# Autodesk Inventor assembly: 脚クランク1
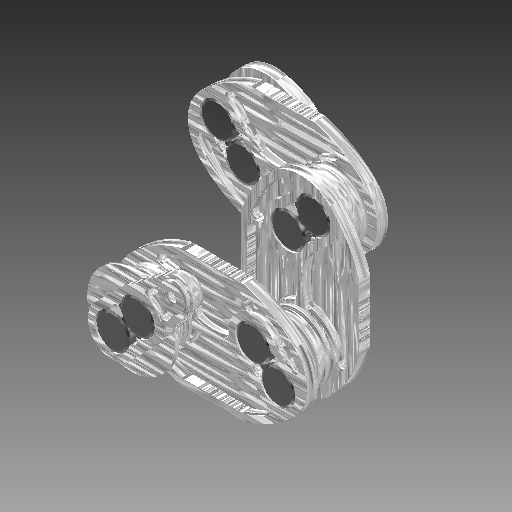
[picture p0: Inventor's stored thumbnail of the model, 512x512]
Saved by Autodesk Inventor 2020 (Build 240168000, 168)
## iProperties
Created: 2019-07-23
Part Number: 脚クランク1
Document SubType Name: Assembly
Designer: 雪村
Mass: 36.597 g
Surface Area: 166.088 cm^2
Volume: 9.97598 cm^3
Density: 3.66852 g/cm^3
Author: 雪村
## Documents named in this file (7)
- C:\Users\white\Documents\SRDC\SRDC\Inventor_2017\2018年機体\2020年4年機体\脚クランク1.iam
- C:\Users\white\Documents\SRDC\SRDC\Inventor_2017\2018年機体\2020年4年機体\脚クランクカム1.ipt
- C:\Users\white\Documents\SRDC\SRDC\Inventor_2017\2018年機体\2020年4年機体\脚クランクハッピーターン1.ipt
- C:\Users\white\Documents\SRDC\SRDC\Inventor_2017\2018年機体\2020年4年機体\脚クランクハッピーターン最終段1.ipt
- C:\Users\white\Documents\SRDC\SRDC\Inventor_2017\2018年機体\2020年4年機体\脚クランク涙型1.ipt
- C:\Users\white\Documents\SRDC\SRDC\Inventor_2017\2018年機体\パーツ\平行ピンΦ2.5,08.ipt
- C:\Users\white\Documents\SRDC\SRDC\Inventor_2017\2018年機体\パーツ\ネジローヘッドm4,08.ipt
## Components (25 placed, 6 different names)
1. 脚クランクカム1:1 — 挿入:5, 挿入:6, 挿入:7, メイト:1
2. 脚クランクハッピーターン1:1 — 挿入:7, メイト:1, 挿入:8, 挿入:9, 挿入:19, 挿入:20, 挿入:25, 挿入:26
3. 脚クランクハッピーターン最終段1:1 — 挿入:1, 挿入:2, 挿入:15, 挿入:16
4. 脚クランク涙型1:1 — 挿入:13, 挿入:14, 挿入:29, 挿入:30
5. 脚クランクハッピーターン1:2 — 挿入:3, 挿入:4, 挿入:5, 挿入:6, 挿入:17, 挿入:18, 挿入:23, 挿入:24
6. 脚クランクハッピーターン1:3 — 挿入:10, メイト:2, 挿入:11, 挿入:12, 挿入:21, 挿入:22, 挿入:27, 挿入:28
7. 脚クランクカム1:2 — 挿入:8, 挿入:9, 挿入:10, メイト:2
8. 脚クランクカム1:3 — 挿入:1, 挿入:2, 挿入:3, 挿入:4
9. 脚クランクカム1:4 — 挿入:11, 挿入:12, 挿入:13, 挿入:14
10. 平行ピンΦ2.5,08:1 — 挿入:17
11. 平行ピンΦ2.5,08:2 — 挿入:16
12. 平行ピンΦ2.5,08:3 — 挿入:15
13. 平行ピンΦ2.5,08:4 — 挿入:18
14. 平行ピンΦ2.5,08:5 — 挿入:19
15. 平行ピンΦ2.5,08:6 — 挿入:20
16. 平行ピンΦ2.5,08:7 — 挿入:21
17. 平行ピンΦ2.5,08:8 — 挿入:22
18. ネジローヘッドm4,08:1 — 挿入:30
19. ネジローヘッドm4,08:2 — 挿入:29
20. ネジローヘッドm4,08:3 — 挿入:28
21. ネジローヘッドm4,08:4 — 挿入:27
22. ネジローヘッドm4,08:5 — 挿入:26
23. ネジローヘッドm4,08:6 — 挿入:25
24. ネジローヘッドm4,08:7 — 挿入:24
25. ネジローヘッドm4,08:8 — 挿入:23
## Relationships (32: Insert 30, Mate 2)
- 挿入:1 [Insert]: 脚クランクハッピーターン最終段1:1 ↔ 脚クランクカム1:3
- 挿入:2 [Insert]: 脚クランクハッピーターン最終段1:1 ↔ 脚クランクカム1:3
- 挿入:3 [Insert]: 脚クランクハッピーターン1:2 ↔ 脚クランクカム1:3
- 挿入:4 [Insert]: 脚クランクハッピーターン1:2 ↔ 脚クランクカム1:3
- 挿入:5 [Insert]: 脚クランクカム1:1 ↔ 脚クランクハッピーターン1:2
- 挿入:6 [Insert]: 脚クランクカム1:1 ↔ 脚クランクハッピーターン1:2
- 挿入:7 [Insert]: 脚クランクカム1:1 ↔ 脚クランクハッピーターン1:1
- メイト:1 [Mate]: 脚クランクカム1:1 ↔ 脚クランクハッピーターン1:1
- 挿入:8 [Insert]: 脚クランクハッピーターン1:1 ↔ 脚クランクカム1:2
- 挿入:9 [Insert]: 脚クランクハッピーターン1:1 ↔ 脚クランクカム1:2
- 挿入:10 [Insert]: 脚クランクハッピーターン1:3 ↔ 脚クランクカム1:2
- メイト:2 [Mate]: 脚クランクハッピーターン1:3 ↔ 脚クランクカム1:2
- 挿入:11 [Insert]: 脚クランクハッピーターン1:3 ↔ 脚クランクカム1:4
- 挿入:12 [Insert]: 脚クランクハッピーターン1:3 ↔ 脚クランクカム1:4
- 挿入:13 [Insert]: 脚クランク涙型1:1 ↔ 脚クランクカム1:4
- 挿入:14 [Insert]: 脚クランク涙型1:1 ↔ 脚クランクカム1:4
- 挿入:15 [Insert]: 脚クランクハッピーターン最終段1:1 ↔ 平行ピンΦ2.5,08:3
- 挿入:16 [Insert]: 脚クランクハッピーターン最終段1:1 ↔ 平行ピンΦ2.5,08:2
- 挿入:17 [Insert]: 脚クランクハッピーターン1:2 ↔ 平行ピンΦ2.5,08:1
- 挿入:18 [Insert]: 脚クランクハッピーターン1:2 ↔ 平行ピンΦ2.5,08:4
- 挿入:19 [Insert]: 脚クランクハッピーターン1:1 ↔ 平行ピンΦ2.5,08:5
- 挿入:20 [Insert]: 脚クランクハッピーターン1:1 ↔ 平行ピンΦ2.5,08:6
- 挿入:21 [Insert]: 脚クランクハッピーターン1:3 ↔ 平行ピンΦ2.5,08:7
- 挿入:22 [Insert]: 脚クランクハッピーターン1:3 ↔ 平行ピンΦ2.5,08:8
- 挿入:23 [Insert]: 脚クランクハッピーターン1:2 ↔ ネジローヘッドm4,08:8
- 挿入:24 [Insert]: 脚クランクハッピーターン1:2 ↔ ネジローヘッドm4,08:7
- 挿入:25 [Insert]: 脚クランクハッピーターン1:1 ↔ ネジローヘッドm4,08:6
- 挿入:26 [Insert]: 脚クランクハッピーターン1:1 ↔ ネジローヘッドm4,08:5
- 挿入:27 [Insert]: 脚クランクハッピーターン1:3 ↔ ネジローヘッドm4,08:4
- 挿入:28 [Insert]: 脚クランクハッピーターン1:3 ↔ ネジローヘッドm4,08:3
- 挿入:29 [Insert]: 脚クランク涙型1:1 ↔ ネジローヘッドm4,08:2
- 挿入:30 [Insert]: 脚クランク涙型1:1 ↔ ネジローヘッドm4,08:1
